# Autodesk Inventor assembly: GearBox
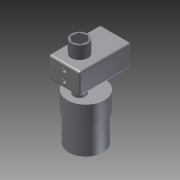
[picture p0: Inventor's stored thumbnail of the model, 180x180]
Saved by Autodesk Inventor 2012 (Build 160160000, 160)
## iProperties
Created: 2011-10-22
Part Number: GearBox
Document SubType Name: Assembly
Designer: KuttaA
Author: KuttaA
## Documents named in this file (8)
- C:\Users\KuttaA\Dropbox\Hexapod Research\Leg Design\Other Parts\Intermediary Gear Box\GearBox.iam
- C:\Users\KuttaA\Dropbox\Hexapod Research\Leg Design\Other Parts\Motor.ipt
- C:\Users\KuttaA\Dropbox\Hexapod Research\Leg Design\Other Parts\GearLargeAndSmall.ipt
- C:\Users\KuttaA\Dropbox\Hexapod Research\Leg Design\Other Parts\Intermediary Gear Box\LargeGearMotorInput.ipt
- C:\Users\KuttaA\Dropbox\Hexapod Research\Leg Design\Other Parts\Intermediary Gear Box\SmallGearOutput.ipt
- C:\Users\KuttaA\Dropbox\Hexapod Research\Leg Design\Other Parts\Intermediary Gear Box\LargeSmallGearAxis.ipt
- C:\Users\KuttaA\Dropbox\Hexapod Research\Leg Design\Other Parts\Intermediary Gear Box\GearboxWallOutput.ipt
- C:\Users\KuttaA\Dropbox\Hexapod Research\Leg Design\Other Parts\Intermediary Gear Box\GearBoxTop.ipt
## Components (7 placed, 7 different names)
1. Motor:1 — Mate:1, Tangent:1, Flush:1, Tangent:2, Mate:2
2. GearLargeAndSmall:1 — Flush:2, Rotation:1, Flush:3, Mate:2, Flush:4
3. LargeGearMotorInput:1 — Mate:1, Tangent:1, Flush:1, Flush:2, Rotation:1, Flush:8, Flush:10
4. Spur Gear1:1 — Flush:3, Tangent:2, Flush:9
5. LargeSmallGearAxis:1 — Flush:4, Angle:1, Flush:5
6. GearboxWallOutput:1 — Flush:5, Flush:6, Flush:7, Flush:8, Flush:9
7. GearBoxTop:1 — Flush:6, Flush:7
## Relationships (16: Flush 10, Mate 2, Tangent 2, RelateRotation 1, Angle 1)
- Mate:1 (0.3 mm): Motor:1 ↔ LargeGearMotorInput:1
- Tangent:1: Motor:1 ↔ LargeGearMotorInput:1
- Flush:1: Motor:1 ↔ LargeGearMotorInput:1
- Flush:2: GearLargeAndSmall:1 ↔ LargeGearMotorInput:1
- Rotation:1 [RelateRotation] (1.4142 ul): GearLargeAndSmall:1 ↔ LargeGearMotorInput:1
- Flush:3: GearLargeAndSmall:1 ↔ Spur Gear1:1
- Tangent:2 (-0.5 mm): Motor:1 ↔ Spur Gear1:1
- Mate:2: Motor:1 ↔ GearLargeAndSmall:1
- Flush:4: GearLargeAndSmall:1 ↔ LargeSmallGearAxis:1
- Angle:1 (0 deg): LargeSmallGearAxis:1
- Flush:5: LargeSmallGearAxis:1 ↔ GearboxWallOutput:1
- Flush:6: GearboxWallOutput:1 ↔ GearBoxTop:1
- Flush:7: GearboxWallOutput:1 ↔ GearBoxTop:1
- Flush:8: LargeGearMotorInput:1 ↔ GearboxWallOutput:1
- Flush:9: Spur Gear1:1 ↔ GearboxWallOutput:1
- Flush:10: LargeGearMotorInput:1
